# Autodesk Inventor assembly: prednja_strana_vrata_sa_ormarom
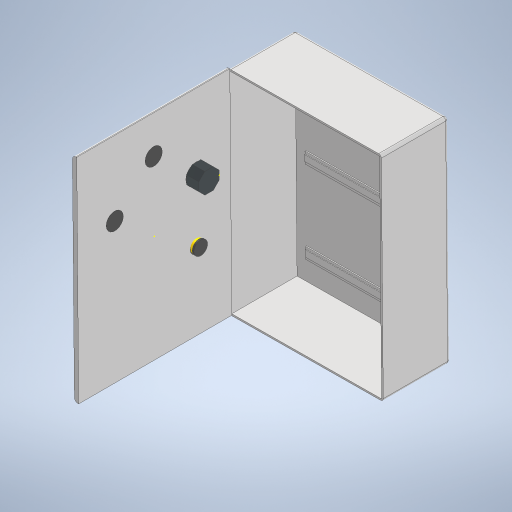
[picture p0: Inventor's stored thumbnail of the model, 512x512]
Saved by Autodesk Inventor 2023 (Build 270158000, 158)
## iProperties
Created: 2022-07-17
Part Number: prednja_strana_vrata_sa_ormarom
Document SubType Name: Assembly
Designer: User
Author: User
## Documents named in this file (3)
- C:\Users\User\Desktop\PMS\Seminarski rad\Inventor_sheme\prednja_strana_vrata_sa_ormarom.iam
- C:\Users\User\Desktop\PMS\Seminarski rad\Inventor_sheme\Ormar.ipt
- C:\Users\User\Desktop\PMS\Seminarski rad\Inventor_sheme\Prednja_strana_vrata.iam
## Components (2 placed, 2 different names)
1. Ormar:1 — Mate:1
2. Prednja_strana_vrata:1 [sub-assembly] — Mate:1
## Relationships (1: Mate 1)
- Mate:1: Ormar:1 ↔ Prednja_strana_vrata:1
